# Autodesk Inventor assembly: Ensamblaje1
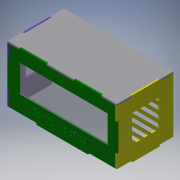
[picture p0: Inventor's stored thumbnail of the model, 180x180]
Saved by Autodesk Inventor 2018 (Build 220112000, 112)
## iProperties
Created: 2020-03-09
Part Number: Ensamblaje1
Material: Genérico
Document SubType Name: Assembly
Designer: joser
Author: joser
## Documents named in this file (6)
- C:\Users\joser\OneDrive\Documentos\UVG\2020\Digital 2\Proyecto\Maqueta\Ensamblaje1.iam
- C:\Users\joser\OneDrive\Documentos\UVG\2020\Digital 2\Proyecto\Maqueta\Control techo.ipt
- C:\Users\joser\OneDrive\Documentos\UVG\2020\Digital 2\Proyecto\Maqueta\Control Frontal.ipt
- C:\Users\joser\OneDrive\Documentos\UVG\2020\Digital 2\Proyecto\Maqueta\Control lateral.ipt
- C:\Users\joser\OneDrive\Documentos\UVG\2020\Digital 2\Proyecto\Maqueta\Control lateral ventilador.ipt
- C:\Users\joser\OneDrive\Documentos\UVG\2020\Digital 2\Proyecto\Maqueta\Vidrio.ipt
## Components (5 placed, 5 different names)
1. Control techo:1 — Coincidencia:1, Coincidencia:2, Coincidencia:3, Coincidencia:4, Coincidencia:6, Coincidencia:7, Coincidencia:8
2. Control Frontal:1 — Coincidencia:1, Coincidencia:2, Coincidencia:3, Coincidencia:5, Coincidencia:9, Coincidencia:10, Coincidencia:11, Nivelación:1
3. Control lateral:1 — Coincidencia:4, Coincidencia:5, Coincidencia:6
4. Control lateral ventilador:1 — Coincidencia:7, Coincidencia:8, Coincidencia:9
5. Vidrio:1 — Coincidencia:10, Coincidencia:11, Nivelación:1
## Relationships (12: Mate 11, Flush 1)
- Coincidencia:1 [Mate]: Control techo:1 ↔ Control Frontal:1
- Coincidencia:2 [Mate]: Control techo:1 ↔ Control Frontal:1
- Coincidencia:3 [Mate]: Control techo:1 ↔ Control Frontal:1
- Coincidencia:4 [Mate]: Control techo:1 ↔ Control lateral:1
- Coincidencia:5 [Mate]: Control Frontal:1 ↔ Control lateral:1
- Coincidencia:6 [Mate]: Control techo:1 ↔ Control lateral:1
- Coincidencia:7 [Mate]: Control techo:1 ↔ Control lateral ventilador:1
- Coincidencia:8 [Mate]: Control techo:1 ↔ Control lateral ventilador:1
- Coincidencia:9 [Mate]: Control Frontal:1 ↔ Control lateral ventilador:1
- Coincidencia:10 [Mate]: Control Frontal:1 ↔ Vidrio:1
- Coincidencia:11 [Mate]: Control Frontal:1 ↔ Vidrio:1
- Nivelación:1 [Flush]: Control Frontal:1 ↔ Vidrio:1
